# Autodesk Inventor assembly: kamera gesamt
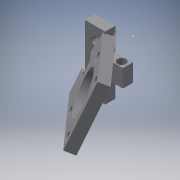
[picture p0: Inventor's stored thumbnail of the model, 180x180]
Saved by Autodesk Inventor 2018 (Build 220112000, 112)
## iProperties
Created: 2018-01-30
Part Number: kamera gesamt
Material: Generisch
Document SubType Name: Assembly
Designer: Andreas
Author: Andreas
## Documents named in this file (3)
- C:\Users\Chris\OneDrive\Development\RTW\03_Konstruktion\kamera gesamt.iam
- C:\Users\Chris\OneDrive\Development\RTW\03_Konstruktion\kamera ot.ipt
- C:\Users\Chris\OneDrive\Development\RTW\03_Konstruktion\kamera ut.ipt
## Components (2 placed, 2 different names)
1. kamera ot:1 — Passend:1
2. kamera ut:1 — Passend:1
## Relationships (1: Mate 1)
- Passend:1 [Mate]: kamera ot:1 ↔ kamera ut:1
